# Autodesk Inventor assembly: Zespół1
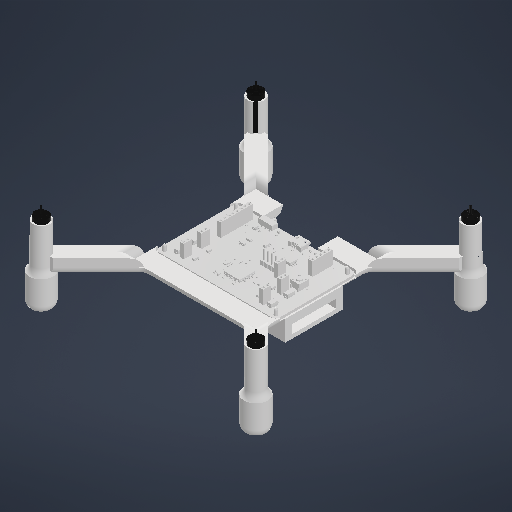
[picture p0: Inventor's stored thumbnail of the model, 512x512]
Saved by Autodesk Inventor 2026 (Build 300175050, 175E)
## iProperties
Created: 2026-01-10
Part Number: Zespół1
Document SubType Name: Assembly
Designer: DeathLock
Author: DeathLock
## Documents named in this file (4)
- C:\Users\DeathLock\Desktop\Zespół1.iam
- C:\Users\DeathLock\Desktop\8520 Coreless Brshed motor.ipt
- C:\Users\DeathLock\Desktop\Drone.ipt
- C:\Users\DeathLock\Desktop\Drone_PCB.ipt
## Components (6 placed, 3 different names)
1. Drone:1 — Sztywne:1, Sztywne:2, Sztywne:3, Sztywne:4, Sztywne:5
2. Drone_PCB:1 — Sztywne:1
3. 8520 Coreless Brshed motor:1 — Sztywne:3
4. 8520 Coreless Brshed motor:2 — Sztywne:4
5. 8520 Coreless Brshed motor:3 — Sztywne:5
6. 8520 Coreless Brshed motor:4 — Sztywne:2
## Relationships (5: WeldJoint 5)
- Sztywne:1 [WeldJoint]: Drone:1 ↔ Drone_PCB:1
- Sztywne:2 [WeldJoint]: Drone:1 ↔ 8520 Coreless Brshed motor:4
- Sztywne:3 [WeldJoint]: Drone:1 ↔ 8520 Coreless Brshed motor:1
- Sztywne:4 [WeldJoint]: Drone:1 ↔ 8520 Coreless Brshed motor:2
- Sztywne:5 [WeldJoint]: Drone:1 ↔ 8520 Coreless Brshed motor:3
